# Autodesk Inventor assembly: Main
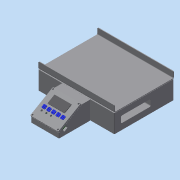
[picture p0: Inventor's stored thumbnail of the model, 180x180]
Saved by Autodesk Inventor 2018 (Build 220112000, 112)
## iProperties
Created: 2020-10-03
Part Number: Main
Material: Generisch
Document SubType Name: Assembly
Designer: marce
Author: marce
## Documents named in this file (14)
- C:\Users\marce\Documents\Waage\CAD\Main.iam
- C:\Users\marce\Documents\Waage\CAD\Schiled.ipt
- C:\Users\marce\Documents\Waage\CAD\Gehause.ipt
- C:\Users\marce\Documents\Waage\CAD\Unterlagscheibe.ipt
- C:\Users\marce\Documents\Waage\CAD\LCD_Distanz.ipt
- C:\Users\marce\Documents\Waage\CAD\Hauptplatte.ipt
- C:\Users\marce\Documents\Waage\CAD\LoadCell.ipt
- C:\Users\marce\Documents\Waage\CAD\Schale.ipt
- C:\Users\marce\Documents\Waage\CAD\PCB\WaagePCB.ipt
- C:\Users\marce\Documents\Waage\CAD\Taster_B.ipt
- C:\Users\marce\Documents\Waage\CAD\Taster_P.ipt
- C:\Users\marce\Documents\Waage\CAD\Taster_Summe.ipt
- C:\Users\marce\Documents\Waage\CAD\Taster_Total.ipt
- C:\Users\marce\Documents\Waage\CAD\Taster_Erase.ipt
## Components (21 placed, 13 different names)
1. WaagePCB:1 — Passend:58, Passend:65, Passend:66, Passend:67, Passend:68, Passend:69, Passend:70, Passend:71, Passend:72, Passend:73, Passend:74
2. Schiled:1 — Passend:4, Passend:7, Passend:14, Passend:16, Passend:17, Passend:19, Fluchtend:1, Passend:20, Passend:29, Passend:30, Passend:32, Passend:33, Passend:34, Passend:35, Passend:36, Passend:79, Passend:80
3. Taster_Summe:1 — Passend:16, Passend:32, Passend:33
4. Taster_Erase:1 — Passend:4, Passend:36, Passend:73
5. Taster_Total:1 — Passend:7, Passend:17, Passend:34, Passend:35
6. Taster_P:1 — Passend:29, Passend:30, Passend:74
7. Taster_B:1 — Passend:14, Passend:79, Passend:80
8. Gehause:1 — Passend:19, Fluchtend:1, Passend:20, Passend:21, Passend:22, Passend:46, Fluchtend:4, Fluchtend:5, Passend:59, Passend:60, Passend:61, Passend:62, Passend:63, Passend:64, Passend:75, Passend:76, Passend:77, Passend:78
9. Unterlagscheibe:1 — Passend:59, Passend:60
10. Unterlagscheibe:2 — Passend:58, Passend:61, Passend:64
11. Unterlagscheibe:3 — Passend:22, Passend:63
12. Unterlagscheibe:4 — Passend:21, Passend:62
13. LCD_Distanz:1 — Passend:71, Passend:72
14. LCD_Distanz:2 — Passend:69, Passend:70
15. LCD_Distanz:3 — Passend:65, Passend:66
16. LCD_Distanz:4 — Passend:67, Passend:68
17. Hauptplatte:1 — Passend:46, Fluchtend:4, Fluchtend:5, Passend:47, Passend:48, Passend:49, Passend:50, Passend:51, Passend:52, Passend:53, Passend:54, Passend:55, Fluchtend:6, Fluchtend:7, Passend:57, Passend:75, Passend:76, Passend:77, Passend:78
18. LoadCell:1 — Passend:47, Passend:48, Passend:49
19. LoadCell:2 — Passend:50, Passend:54, Passend:55
20. LoadCell:3 — Passend:51, Passend:52, Passend:53, Passend:56
21. Schale:1 — Passend:56, Fluchtend:6, Fluchtend:7
## Relationships (56: Mate 51, Flush 5)
- Passend:4 [Mate]: Schiled:1 ↔ Taster_Erase:1
- Passend:7 [Mate]: Schiled:1 ↔ Taster_Total:1
- Passend:14 [Mate]: Schiled:1 ↔ Taster_B:1
- Passend:16 [Mate]: Schiled:1 ↔ Taster_Summe:1
- Passend:17 [Mate]: Schiled:1 ↔ Taster_Total:1
- Passend:19 [Mate]: Schiled:1 ↔ Gehause:1
- Fluchtend:1 [Flush]: Schiled:1 ↔ Gehause:1
- Passend:20 [Mate]: Schiled:1 ↔ Gehause:1
- Passend:21 [Mate]: Gehause:1 ↔ Unterlagscheibe:4
- Passend:22 [Mate]: Gehause:1 ↔ Unterlagscheibe:3
- Passend:29 [Mate]: Schiled:1 ↔ Taster_P:1
- Passend:30 [Mate]: Schiled:1 ↔ Taster_P:1
- Passend:32 [Mate]: Schiled:1 ↔ Taster_Summe:1
- Passend:33 [Mate]: Schiled:1 ↔ Taster_Summe:1
- Passend:34 [Mate]: Schiled:1 ↔ Taster_Total:1
- Passend:35 [Mate]: Schiled:1 ↔ Taster_Total:1
- Passend:36 [Mate]: Schiled:1 ↔ Taster_Erase:1
- Passend:46 [Mate]: Gehause:1 ↔ Hauptplatte:1
- Fluchtend:4 [Flush]: Gehause:1 ↔ Hauptplatte:1
- Fluchtend:5 [Flush] (-72.5 mm): Gehause:1 ↔ Hauptplatte:1
- Passend:47 [Mate]: Hauptplatte:1 ↔ LoadCell:1
- Passend:48 [Mate]: Hauptplatte:1 ↔ LoadCell:1
- Passend:49 [Mate]: Hauptplatte:1 ↔ LoadCell:1
- Passend:50 [Mate]: Hauptplatte:1 ↔ LoadCell:2
- Passend:51 [Mate]: Hauptplatte:1 ↔ LoadCell:3
- Passend:52 [Mate]: Hauptplatte:1 ↔ LoadCell:3
- Passend:53 [Mate]: Hauptplatte:1 ↔ LoadCell:3
- Passend:54 [Mate]: Hauptplatte:1 ↔ LoadCell:2
- Passend:55 [Mate]: Hauptplatte:1 ↔ LoadCell:2
- Passend:56 [Mate] (2 mm): LoadCell:3 ↔ Schale:1
- Fluchtend:6 [Flush]: Hauptplatte:1 ↔ Schale:1
- Fluchtend:7 [Flush]: Hauptplatte:1 ↔ Schale:1
- Passend:57 [Mate]: Hauptplatte:1
- Passend:58 [Mate]: WaagePCB:1 ↔ Unterlagscheibe:2
- Passend:59 [Mate]: Gehause:1 ↔ Unterlagscheibe:1
- Passend:60 [Mate]: Gehause:1 ↔ Unterlagscheibe:1
- Passend:61 [Mate]: Gehause:1 ↔ Unterlagscheibe:2
- Passend:62 [Mate]: Gehause:1 ↔ Unterlagscheibe:4
- Passend:63 [Mate]: Gehause:1 ↔ Unterlagscheibe:3
- Passend:64 [Mate]: Gehause:1 ↔ Unterlagscheibe:2
- Passend:65 [Mate]: WaagePCB:1 ↔ LCD_Distanz:3
- Passend:66 [Mate]: WaagePCB:1 ↔ LCD_Distanz:3
- Passend:67 [Mate]: WaagePCB:1 ↔ LCD_Distanz:4
- Passend:68 [Mate]: WaagePCB:1 ↔ LCD_Distanz:4
- Passend:69 [Mate]: WaagePCB:1 ↔ LCD_Distanz:2
- Passend:70 [Mate]: WaagePCB:1 ↔ LCD_Distanz:2
- Passend:71 [Mate]: WaagePCB:1 ↔ LCD_Distanz:1
- Passend:72 [Mate]: WaagePCB:1 ↔ LCD_Distanz:1
- Passend:73 [Mate]: WaagePCB:1 ↔ Taster_Erase:1
- Passend:74 [Mate]: WaagePCB:1 ↔ Taster_P:1
- Passend:75 [Mate]: Gehause:1 ↔ Hauptplatte:1
- Passend:76 [Mate]: Gehause:1 ↔ Hauptplatte:1
- Passend:77 [Mate]: Gehause:1 ↔ Hauptplatte:1
- Passend:78 [Mate]: Gehause:1 ↔ Hauptplatte:1
- Passend:79 [Mate]: Schiled:1 ↔ Taster_B:1
- Passend:80 [Mate]: Schiled:1 ↔ Taster_B:1
